# Autodesk Inventor assembly: VersaPlanetary All Non-CIM Motors_NeveRest Motor
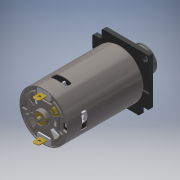
[picture p0: Inventor's stored thumbnail of the model, 180x180]
Saved by Autodesk Inventor 2018 (Build 220112000, 112)
## iProperties
Created: 2020-02-03
Part Number: VersaPlanetary All Non-CIM Motors_NeveRest Motor
Document SubType Name: Assembly
Designer: maste
Author: maste
Revision Number: ANY
## Documents named in this file (9)
- C:\Users\maste\OneDrive\Documents\GitHub\2020CAD\Control panel spinny boi\Part Files\VersaPlanetary All Non-CIM Motors_NeveRest Motor.iam
- C:\Users\maste\OneDrive\Documents\GitHub\2020CAD\Control panel spinny boi\Part Files\am-3104.iam
- C:\Users\maste\OneDrive\Documents\GitHub\2020CAD\Control panel spinny boi\Part Files\217-2625-012 Rev1.ipt
- C:\Users\maste\OneDrive\Documents\GitHub\2020CAD\Control panel spinny boi\Part Files\217-4649-001 Rev1.ipt
- C:\Users\maste\OneDrive\Documents\GitHub\2020CAD\Control panel spinny boi\Part Files\217-4649-007 Rev1_94105A824.ipt
- C:\Users\maste\OneDrive\Documents\GitHub\2020CAD\Control panel spinny boi\Part Files\217-2822-001 Rev4.ipt
- C:\Users\maste\OneDrive\Documents\GitHub\2020CAD\Control panel spinny boi\Part Files\217-4649-005 Rev1_SSA0003-008BA.ipt
- C:\Users\maste\OneDrive\Documents\GitHub\2020CAD\Control panel spinny boi\Part Files\217-4649-006 Rev1_SSA0004-008BA.ipt
- C:\Users\maste\OneDrive\Documents\GitHub\2020CAD\Control panel spinny boi\Part Files\RS550 12V DC Motor.iam
## Components (9 placed, 9 different names)
1. am-3104_10 [sub-assembly]
2. 217-2625-012 Rev1_11
3. 217-4649-001 Rev1_12
4. 217-4649-007 Rev1_94105A824_13
5. 217-2822-001 Rev4_14 — Mate:3
6. 217-4649-005 Rev1_SSA0003-008BA_15 — Mate:2
7. 217-4649-005 Rev1_SSA0003-008BA_16
8. 217-4649-006 Rev1_SSA0004-008BA_17 — Mate:1
9. RS550 12V DC Motor:1 [sub-assembly] — Mate:1, Mate:2, Mate:3
## Relationships (3: Mate 3)
- Mate:1: 217-4649-006 Rev1_SSA0004-008BA_17 ↔ RS550 12V DC Motor:1
- Mate:2: 217-4649-005 Rev1_SSA0003-008BA_15 ↔ RS550 12V DC Motor:1
- Mate:3: 217-2822-001 Rev4_14 ↔ RS550 12V DC Motor:1
